# Autodesk Inventor assembly: E-Chassis_Assemly
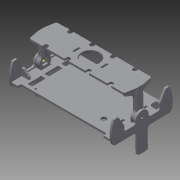
[picture p0: Inventor's stored thumbnail of the model, 180x180]
Saved by Autodesk Inventor 2015 (Build 190159000, 159)
## iProperties
Created: 2015-08-05
Part Number: E-Chassis_Assemly
Document SubType Name: Assembly
Designer: Thomas
Author: Thomas
## Documents named in this file (7)
- C:\Users\Thomas\Google Drive\MSc ROBOTICS\PROJECT\OpenROV\openrov-hardware\CAD_Files_OpenROV_v2_5\E-Chassis_Assemly.iam
- C:\Users\Thomas\Google Drive\MSc ROBOTICS\PROJECT\OpenROV\openrov-hardware\CAD_Files_OpenROV_v2_5\E-Chassis\Main_Platform.ipt
- C:\Users\Thomas\Google Drive\MSc ROBOTICS\PROJECT\OpenROV\openrov-hardware\CAD_Files_OpenROV_v2_5\E-Chassis\Endplate.ipt
- C:\Users\Thomas\Google Drive\MSc ROBOTICS\PROJECT\OpenROV\openrov-hardware\CAD_Files_OpenROV_v2_5\E-Chassis\Endplate_Support.ipt
- C:\Users\Thomas\Google Drive\MSc ROBOTICS\PROJECT\OpenROV\openrov-hardware\CAD_Files_OpenROV_v2_5\E-Chassis\Camera_Mount_A.ipt
- C:\Users\Thomas\Google Drive\MSc ROBOTICS\PROJECT\OpenROV\openrov-hardware\CAD_Files_OpenROV_v2_5\E-Chassis\Camera_Mount_B.ipt
- C:\Users\Thomas\Google Drive\MSc ROBOTICS\PROJECT\OpenROV\openrov-hardware\CAD_Files_OpenROV_v2_5\E-Chassis\Camera_Platform.ipt
## Components (12 placed, 6 different names)
1. Main_Platform:1
2. Endplate:1
3. Endplate:2
4. Endplate_Support:1
5. Endplate_Support:2
6. Endplate_Support:3
7. Endplate_Support:4
8. Camera_Mount_A:1
9. Camera_Mount_A:2
10. Camera_Mount_B:1
11. Camera_Mount_B:2
12. Camera_Platform:1
## Relationships (31: Mate 29, Flush 2)
- [Mate]: Main_Platform:1 ↔ Endplate:1
- [Mate]: Main_Platform:1 ↔ Endplate:1
- [Mate]: Main_Platform:1 ↔ Endplate:1
- [Mate]: Main_Platform:1 ↔ Endplate:2
- [Mate]: Main_Platform:1 ↔ Endplate:2
- [Mate]: Main_Platform:1 ↔ Endplate:2
- [Mate]: Endplate:1 ↔ Endplate_Support:2
- [Mate]: Main_Platform:1 ↔ Endplate_Support:2
- [Mate]: Endplate:1 ↔ Endplate_Support:2
- [Mate]: Endplate:1 ↔ Endplate_Support:1
- [Mate]: Main_Platform:1 ↔ Endplate_Support:1
- [Mate]: Endplate:1 ↔ Endplate_Support:1
- [Mate]: Endplate:2 ↔ Endplate_Support:4
- [Mate]: Main_Platform:1 ↔ Endplate_Support:4
- [Mate]: Endplate:2 ↔ Endplate_Support:4
- [Mate]: Endplate:2 ↔ Endplate_Support:3
- [Mate]: Main_Platform:1 ↔ Endplate_Support:3
- [Mate]: Endplate:2 ↔ Endplate_Support:3
- [Mate]: Camera_Mount_A:2 ↔ Camera_Mount_B:2
- [Mate]: Camera_Mount_A:2 ↔ Camera_Mount_B:2
- [Flush]: Camera_Mount_A:2 ↔ Camera_Mount_B:2
- [Mate]: Camera_Mount_A:1 ↔ Camera_Mount_B:1
- [Mate]: Camera_Mount_A:1 ↔ Camera_Mount_B:1
- [Flush]: Camera_Mount_A:1 ↔ Camera_Mount_B:1
- [Mate]: Endplate:2 ↔ Camera_Mount_A:1
- [Mate]: Endplate:2 ↔ Camera_Mount_A:1
- [Mate]: Endplate:1 ↔ Camera_Mount_A:2
- [Mate]: Endplate:1 ↔ Camera_Mount_A:2
- [Mate]: Camera_Mount_B:1 ↔ Camera_Platform:1
- [Mate]: Camera_Mount_B:1 ↔ Camera_Platform:1
- [Mate]: Camera_Mount_B:2 ↔ Camera_Platform:1
